# Autodesk Inventor assembly: Full Keyboard
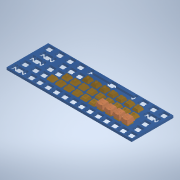
[picture p0: Inventor's stored thumbnail of the model, 180x180]
Saved by Autodesk Inventor 2022 (Build 260153000, 153)
## iProperties
Created: 2022-03-01
Part Number: Full Keyboard
Document SubType Name: Assembly
Designer: Nathan Griffith
Author: Nathan Griffith
## Documents named in this file (7)
- C:\Users\Nathan Griffith\Documents\Inventor\Eric's Keyboard\Full Keyboard.iam
- C:\Users\Nathan Griffith\Documents\Inventor\Eric's Keyboard\plate.ipt
- C:\Users\Nathan Griffith\Documents\Inventor\Eric's Keyboard\cherry mx.ipt
- C:\Users\Nathan Griffith\Documents\Inventor\Eric's Keyboard\Keycap a-z\KeycapQ.ipt
- C:\Users\Nathan Griffith\Documents\Inventor\Eric's Keyboard\Keycap a-z\KeycapW.ipt
- C:\Users\Nathan Griffith\Documents\Inventor\Eric's Keyboard\Keycap a-z\KeycapE.ipt
- C:\Users\Nathan Griffith\Documents\Inventor\Eric's Keyboard\Keycap a-z\KeycapR.ipt
## Components (31 placed, 6 different names)
1. plate:1 — Mate:1, Mate:2, Mate:3, Mate:4, Mate:5
2. KeycapQ:1 — Mate:6
3. KeycapW:1 — Mate:7
4. KeycapE:1 — Mate:8
5. KeycapR:1 — Mate:9
6. cherry mx:1 — Mate:1, Mate:2, Mate:6
7. cherry mx:2 — Mate:7
8. cherry mx:3 — Mate:8
9. cherry mx:4 — Mate:9
10. cherry mx:5
11. cherry mx:6
12. cherry mx:7
13. cherry mx:8
14. cherry mx:9
15. cherry mx:10
16. cherry mx:11 — Mate:3, Mate:4
17. cherry mx:12
18. cherry mx:13
19. cherry mx:14
20. cherry mx:15
21. cherry mx:16
22. cherry mx:17
23. cherry mx:18
24. cherry mx:19
25. cherry mx:20 — Mate:5
26. cherry mx:21
27. cherry mx:22
28. cherry mx:23
29. cherry mx:24
30. cherry mx:25
31. cherry mx:26
## Component patterns: (10 elements, first: cherry mx:1), (9 elements, first: cherry mx:11), (7 elements, first: cherry mx:20)
## Relationships (9: Mate 9)
- Mate:1: plate:1 ↔ cherry mx:1
- Mate:2: plate:1 ↔ cherry mx:1
- Mate:3: plate:1 ↔ cherry mx:11
- Mate:4: plate:1 ↔ cherry mx:11
- Mate:5: plate:1 ↔ cherry mx:20
- Mate:6: KeycapQ:1 ↔ cherry mx:1
- Mate:7: KeycapW:1 ↔ cherry mx:2
- Mate:8: KeycapE:1 ↔ cherry mx:3
- Mate:9: KeycapR:1 ↔ cherry mx:4
